# Autodesk Inventor assembly: MechanumChassis
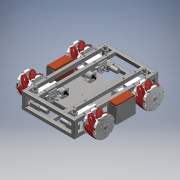
[picture p0: Inventor's stored thumbnail of the model, 180x180]
Saved by Autodesk Inventor 2018 (Build 220112000, 112)
## iProperties
Created: 2017-10-18
Part Number: MechanumChassis
Document SubType Name: Weldment
Designer: Bryce Richards
Mass: 42172.1 g
Surface Area: 44852.8 cm^2
Volume: 5448.29 cm^3
Density: 7.74044 g/cm^3
Weld Material: Steel, Mild, Welded
Author: Bryce Richards
## Documents named in this file (16)
- C:\Users\P136265\Documents\GitHub\mecanum-cad\MechanumChassis.iam
- C:\Users\P136265\Documents\GitHub\mecanum-cad\MecanumFrame2.iam
- C:\Users\P136265\Documents\GitHub\mecanum-cad\WheelShaft.ipt
- C:\Users\P136265\Documents\GitHub\mecanum-cad\Mecanum_Assembly.iam
- C:\Users\P136265\Documents\Inventor\Content Center Files\R2018\en-US\AS 1112 (2)\AS 1112 - M4  Type 5.ipt
- C:\Users\P136265\Documents\GitHub\mecanum-cad\LiftBase.ipt
- C:\Users\P136265\Documents\GitHub\mecanum-cad\BatteryBox_NP1812.ipt
- C:\Users\P136265\Documents\GitHub\mecanum-cad\NP18-12 Battery.ipt
- C:\Users\P136265\Documents\GitHub\mecanum-cad\BearingHousing.iam
- C:\Users\P136265\Documents\Inventor\Content Center Files\R2018\en-US\AS 1110\AS 1110 - M8 x 50.ipt
- C:\Users\P136265\Documents\Inventor\Content Center Files\R2018\en-US\AS 1112 (2)\AS 1112 - M8  Type 5.ipt
- C:\Users\P136265\Documents\GitHub\mecanum-cad\mount.ipt
- C:\Users\P136265\Documents\GitHub\mecanum-cad\Nema 23 Stepper Motor Bipolar L=56mm w Gear Ratio 41 Planetary Gearbox.ipt
- C:\Users\P136265\Documents\GitHub\mecanum-cad\LiftAssembly_Through.iam
- C:\Users\P136265\Documents\Inventor\Content Center Files\R2018\en-US\BS EN 24035\ISO 4035 - M20BS EN.ipt
- C:\Users\P136265\Documents\mecanum-cad\MechanumChassis\AIP\FEA\cayefugld.fres
## Components (78 placed, 14 different names)
1. MecanumFrame2:1 [sub-assembly] — Mate:90, Angle:5, Angle:6, Angle:7, Mate:386, Flush:32, Flush:33, Mate:486, Mate:487, Mate:488, Mate:489, Mate:494, Mate:500, Mate:501, Mate:502, Mate:503, Mate:504, Mate:512, Mate:514, Mate:516, Mate:518, Mate:520, Mate:522, Mate:524, Mate:526, Mate:528, Mate:530, Mate:532, Mate:534, Mate:536, Mate:538, Mate:540, Mate:542, Mate:545, Mate:547, Mate:549, Mate:551, Mate:553, Mate:555, Mate:557, Mate:559, Mate:561, Mate:563, Mate:565, Mate:567, Mate:569, Mate:571, Mate:573, Mate:575, Mate:594, Angle:41, Mate:607, Mate:608, Mate:641, Mate:642, Mate:643, Mate:644, Mate:645, Mate:646, Angle:49, Angle:51
2. Mecanum_Assembly:1 [sub-assembly] — Mate:617, Mate:618, Angle:44, Mate:654
3. Mecanum_Assembly:2 [sub-assembly] — Mate:613, Mate:614, Angle:43, Mate:652
4. Mecanum_Assembly:3 [sub-assembly] — Mate:621, Mate:622, Mate:650
5. Mecanum_Assembly:4 [sub-assembly] — Mate:609, Mate:610, Angle:42, Mate:648
6. LiftBase:1 — Mate:386, Flush:32, Flush:33, Mate:606, Mate:635, Mate:637, Mate:639
7. BatteryBox_NP1812:1 — Mate:459, Mate:461
8. BatteryBox_NP1812:2 — Mate:462, Mate:464
9. NP18-12 Battery:1 — Mate:459, Mate:461, Angle:45, Angle:46
10. NP18-12 Battery:2 — Mate:462, Mate:464, Angle:40, Angle:47
11. AS 1112 (2) - Metric M4  Type 5:17
12. AS 1112 (2) - Metric M4  Type 5:18
13. AS 1112 (2) - Metric M4  Type 5:19
14. AS 1112 (2) - Metric M4  Type 5:20
15. AS 1112 (2) - Metric M4  Type 5:21
16. AS 1112 (2) - Metric M4  Type 5:22
17. AS 1112 (2) - Metric M4  Type 5:23
18. AS 1112 (2) - Metric M4  Type 5:24
19. BearingHousing:1 [sub-assembly] — Mate:486, Mate:487, Mate:488, Mate:489, Mate:493, Mate:521, Mate:523, Mate:525, Mate:527, Mate:611, Mate:612, Mate:660
20. BearingHousing:2 [sub-assembly] — Mate:493, Mate:494, Mate:513, Mate:515, Mate:517, Mate:519, Mate:594, Mate:615, Mate:616, Mate:658
21. BearingHousing:3 [sub-assembly] — Mate:503, Mate:504, Mate:529, Mate:531, Mate:533, Mate:535, Mate:623, Mate:624, Mate:662
22. BearingHousing:4 [sub-assembly] — Mate:500, Mate:501, Mate:502, Mate:537, Mate:539, Mate:541, Mate:543, Mate:619, Mate:620, Mate:656
23. AS 1110 - Metric M8 x 50:3 — Mate:512, Mate:513, Mate:558
24. AS 1110 - Metric M8 x 50:4 — Mate:514, Mate:515, Mate:556
25. AS 1110 - Metric M8 x 50:5 — Mate:516, Mate:517, Mate:552
26. AS 1110 - Metric M8 x 50:6 — Mate:518, Mate:519, Mate:554
27. AS 1110 - Metric M8 x 50:7 — Mate:520, Mate:521, Mate:574
28. AS 1110 - Metric M8 x 50:8 — Mate:522, Mate:523, Mate:572
29. AS 1110 - Metric M8 x 50:9 — Mate:524, Mate:525, Mate:568
30. AS 1110 - Metric M8 x 50:10 — Mate:526, Mate:527, Mate:570
31. AS 1110 - Metric M8 x 50:11 — Mate:528, Mate:529, Mate:566
32. AS 1110 - Metric M8 x 50:12 — Mate:530, Mate:531, Mate:562
33. AS 1110 - Metric M8 x 50:13 — Mate:532, Mate:533, Mate:564
34. AS 1110 - Metric M8 x 50:14 — Mate:534, Mate:535, Mate:560
35. AS 1110 - Metric M8 x 50:15 — Mate:536, Mate:537, Mate:544
36. AS 1110 - Metric M8 x 50:16 — Mate:538, Mate:539, Mate:548
37. AS 1110 - Metric M8 x 50:17 — Mate:540, Mate:541, Mate:546
38. AS 1110 - Metric M8 x 50:18 — Mate:542, Mate:543, Mate:550
39. AS 1112 (2) - Metric M8  Type 5:1 — Mate:544, Mate:545
40. AS 1112 (2) - Metric M8  Type 5:2 — Mate:546, Mate:547
41. AS 1112 (2) - Metric M8  Type 5:3 — Mate:548, Mate:549
42. AS 1112 (2) - Metric M8  Type 5:4 — Mate:550, Mate:551
43. AS 1112 (2) - Metric M8  Type 5:5 — Mate:552, Mate:553
44. AS 1112 (2) - Metric M8  Type 5:6 — Mate:554, Mate:555
45. AS 1112 (2) - Metric M8  Type 5:7 — Mate:556, Mate:557
46. AS 1112 (2) - Metric M8  Type 5:8 — Mate:558, Mate:559
47. AS 1112 (2) - Metric M8  Type 5:9 — Mate:560, Mate:561
48. AS 1112 (2) - Metric M8  Type 5:10 — Mate:562, Mate:563
49. AS 1112 (2) - Metric M8  Type 5:11 — Mate:564, Mate:565
50. AS 1112 (2) - Metric M8  Type 5:12 — Mate:566, Mate:567
51. AS 1112 (2) - Metric M8  Type 5:13 — Mate:568, Mate:569
52. AS 1112 (2) - Metric M8  Type 5:14 — Mate:570, Mate:571
53. AS 1112 (2) - Metric M8  Type 5:15 — Mate:572, Mate:573
54. AS 1112 (2) - Metric M8  Type 5:16 — Mate:574, Mate:575
55. mount:1 — Mate:603, Mate:604, Mate:605, Mate:606
56. Nema 23 Stepper Motor Bipolar L=56mm w Gear Ratio 41 Planetary Gearbox:1 — Mate:603, Mate:604, Mate:605, Angle:40, Angle:41, Flush:34, Mate:625
57. LiftAssembly_Through:1 [sub-assembly] — Mate:607, Mate:608, Angle:48
58. WheelShaft:1 — Mate:621, Mate:622, Mate:623, Mate:624, Flush:37, Mate:640, Mate:649, Mate:661
59. WheelShaft:2 — Mate:617, Mate:618, Mate:619, Mate:620, Angle:44, Flush:36, Mate:638, Mate:653, Mate:655
60. WheelShaft:3 — Mate:613, Mate:614, Mate:615, Mate:616, Angle:43, Flush:35, Mate:636, Mate:651, Mate:657
61. WheelShaft:4 — Mate:609, Mate:610, Angle:42, Mate:611, Mate:612, Flush:34, Mate:625, Mate:647, Mate:659
62. mount:2 — Mate:626, Mate:627, Mate:628, Mate:637
63. mount:3 — Mate:629, Mate:630, Mate:631, Mate:639
64. mount:4 — Mate:632, Mate:633, Mate:634, Mate:635
65. Nema 23 Stepper Motor Bipolar L=56mm w Gear Ratio 41 Planetary Gearbox:2 — Mate:626, Mate:627, Mate:628, Angle:46, Flush:36, Mate:638
66. Nema 23 Stepper Motor Bipolar L=56mm w Gear Ratio 41 Planetary Gearbox:3 — Mate:629, Mate:630, Mate:631, Angle:47, Flush:37, Mate:640
67. Nema 23 Stepper Motor Bipolar L=56mm w Gear Ratio 41 Planetary Gearbox:4 — Mate:632, Mate:633, Mate:634, Angle:45, Flush:35, Mate:636
68. LiftAssembly_Through:2 [sub-assembly] — Mate:641, Mate:642, Angle:50, Angle:51
69. LiftAssembly_Through:3 [sub-assembly] — Mate:643, Mate:644, Angle:50
70. LiftAssembly_Through:4 [sub-assembly] — Mate:645, Mate:646, Angle:48, Angle:49
71. BS EN 24035 - Metric M20:1 — Mate:647, Mate:648
72. BS EN 24035 - Metric M20:2 — Mate:649, Mate:650
73. BS EN 24035 - Metric M20:3 — Mate:651, Mate:652
74. BS EN 24035 - Metric M20:4 — Mate:653, Mate:654
75. BS EN 24035 - Metric M20:5 — Mate:655, Mate:656
76. BS EN 24035 - Metric M20:6 — Mate:657, Mate:658
77. BS EN 24035 - Metric M20:7 — Mate:659, Mate:660
78. BS EN 24035 - Metric M20:8 — Mate:661, Mate:662
## Relationships (163: Mate 142, Angle 15, Flush 6)
- Mate:90: MecanumFrame2:1
- Angle:5 (0 deg): MecanumFrame2:1
- Angle:6 (0 deg): MecanumFrame2:1
- Angle:7 (0 deg): MecanumFrame2:1
- Mate:386: MecanumFrame2:1 ↔ LiftBase:1
- Flush:32 (2.5 mm): MecanumFrame2:1 ↔ LiftBase:1
- Flush:33 (2.5 mm): MecanumFrame2:1 ↔ LiftBase:1
- Mate:459: BatteryBox_NP1812:1 ↔ NP18-12 Battery:1
- Mate:461 (2 mm): BatteryBox_NP1812:1 ↔ NP18-12 Battery:1
- Mate:462: BatteryBox_NP1812:2 ↔ NP18-12 Battery:2
- Mate:464 (2 mm): BatteryBox_NP1812:2 ↔ NP18-12 Battery:2
- Mate:486: MecanumFrame2:1 ↔ BearingHousing:1
- Mate:487: MecanumFrame2:1 ↔ BearingHousing:1
- Mate:488: MecanumFrame2:1 ↔ BearingHousing:1
- Mate:489: MecanumFrame2:1 ↔ BearingHousing:1
- Mate:493: BearingHousing:1 ↔ BearingHousing:2
- Mate:494: MecanumFrame2:1 ↔ BearingHousing:2
- Mate:500: MecanumFrame2:1 ↔ BearingHousing:4
- Mate:501: MecanumFrame2:1 ↔ BearingHousing:4
- Mate:502: MecanumFrame2:1 ↔ BearingHousing:4
- Mate:503: MecanumFrame2:1 ↔ BearingHousing:3
- Mate:504: MecanumFrame2:1 ↔ BearingHousing:3
- Mate:512: MecanumFrame2:1 ↔ AS 1110 - Metric M8 x 50:3
- Mate:513: BearingHousing:2 ↔ AS 1110 - Metric M8 x 50:3
- Mate:514: MecanumFrame2:1 ↔ AS 1110 - Metric M8 x 50:4
- Mate:515: BearingHousing:2 ↔ AS 1110 - Metric M8 x 50:4
- Mate:516: MecanumFrame2:1 ↔ AS 1110 - Metric M8 x 50:5
- Mate:517: BearingHousing:2 ↔ AS 1110 - Metric M8 x 50:5
- Mate:518: MecanumFrame2:1 ↔ AS 1110 - Metric M8 x 50:6
- Mate:519: BearingHousing:2 ↔ AS 1110 - Metric M8 x 50:6
- Mate:520: MecanumFrame2:1 ↔ AS 1110 - Metric M8 x 50:7
- Mate:521: BearingHousing:1 ↔ AS 1110 - Metric M8 x 50:7
- Mate:522: MecanumFrame2:1 ↔ AS 1110 - Metric M8 x 50:8
- Mate:523: BearingHousing:1 ↔ AS 1110 - Metric M8 x 50:8
- Mate:524: MecanumFrame2:1 ↔ AS 1110 - Metric M8 x 50:9
- Mate:525: BearingHousing:1 ↔ AS 1110 - Metric M8 x 50:9
- Mate:526: MecanumFrame2:1 ↔ AS 1110 - Metric M8 x 50:10
- Mate:527: BearingHousing:1 ↔ AS 1110 - Metric M8 x 50:10
- Mate:528: MecanumFrame2:1 ↔ AS 1110 - Metric M8 x 50:11
- Mate:529: BearingHousing:3 ↔ AS 1110 - Metric M8 x 50:11
- Mate:530: MecanumFrame2:1 ↔ AS 1110 - Metric M8 x 50:12
- Mate:531: BearingHousing:3 ↔ AS 1110 - Metric M8 x 50:12
- Mate:532: MecanumFrame2:1 ↔ AS 1110 - Metric M8 x 50:13
- Mate:533: BearingHousing:3 ↔ AS 1110 - Metric M8 x 50:13
- Mate:534: MecanumFrame2:1 ↔ AS 1110 - Metric M8 x 50:14
- Mate:535: BearingHousing:3 ↔ AS 1110 - Metric M8 x 50:14
- Mate:536: MecanumFrame2:1 ↔ AS 1110 - Metric M8 x 50:15
- Mate:537: BearingHousing:4 ↔ AS 1110 - Metric M8 x 50:15
- Mate:538: MecanumFrame2:1 ↔ AS 1110 - Metric M8 x 50:16
- Mate:539: BearingHousing:4 ↔ AS 1110 - Metric M8 x 50:16
- Mate:540: MecanumFrame2:1 ↔ AS 1110 - Metric M8 x 50:17
- Mate:541: BearingHousing:4 ↔ AS 1110 - Metric M8 x 50:17
- Mate:542: MecanumFrame2:1 ↔ AS 1110 - Metric M8 x 50:18
- Mate:543: BearingHousing:4 ↔ AS 1110 - Metric M8 x 50:18
- Mate:544: AS 1110 - Metric M8 x 50:15 ↔ AS 1112 (2) - Metric M8  Type 5:1
- Mate:545: MecanumFrame2:1 ↔ AS 1112 (2) - Metric M8  Type 5:1
- Mate:546: AS 1110 - Metric M8 x 50:17 ↔ AS 1112 (2) - Metric M8  Type 5:2
- Mate:547: MecanumFrame2:1 ↔ AS 1112 (2) - Metric M8  Type 5:2
- Mate:548: AS 1110 - Metric M8 x 50:16 ↔ AS 1112 (2) - Metric M8  Type 5:3
- Mate:549: MecanumFrame2:1 ↔ AS 1112 (2) - Metric M8  Type 5:3
- Mate:550: AS 1110 - Metric M8 x 50:18 ↔ AS 1112 (2) - Metric M8  Type 5:4
- Mate:551: MecanumFrame2:1 ↔ AS 1112 (2) - Metric M8  Type 5:4
- Mate:552: AS 1110 - Metric M8 x 50:5 ↔ AS 1112 (2) - Metric M8  Type 5:5
- Mate:553: MecanumFrame2:1 ↔ AS 1112 (2) - Metric M8  Type 5:5
- Mate:554: AS 1110 - Metric M8 x 50:6 ↔ AS 1112 (2) - Metric M8  Type 5:6
- Mate:555: MecanumFrame2:1 ↔ AS 1112 (2) - Metric M8  Type 5:6
- Mate:556: AS 1110 - Metric M8 x 50:4 ↔ AS 1112 (2) - Metric M8  Type 5:7
- Mate:557: MecanumFrame2:1 ↔ AS 1112 (2) - Metric M8  Type 5:7
- Mate:558: AS 1110 - Metric M8 x 50:3 ↔ AS 1112 (2) - Metric M8  Type 5:8
- Mate:559: MecanumFrame2:1 ↔ AS 1112 (2) - Metric M8  Type 5:8
- Mate:560: AS 1110 - Metric M8 x 50:14 ↔ AS 1112 (2) - Metric M8  Type 5:9
- Mate:561: MecanumFrame2:1 ↔ AS 1112 (2) - Metric M8  Type 5:9
- Mate:562: AS 1110 - Metric M8 x 50:12 ↔ AS 1112 (2) - Metric M8  Type 5:10
- Mate:563: MecanumFrame2:1 ↔ AS 1112 (2) - Metric M8  Type 5:10
- Mate:564: AS 1110 - Metric M8 x 50:13 ↔ AS 1112 (2) - Metric M8  Type 5:11
- Mate:565: MecanumFrame2:1 ↔ AS 1112 (2) - Metric M8  Type 5:11
- Mate:566: AS 1110 - Metric M8 x 50:11 ↔ AS 1112 (2) - Metric M8  Type 5:12
- Mate:567: MecanumFrame2:1 ↔ AS 1112 (2) - Metric M8  Type 5:12
- Mate:568: AS 1110 - Metric M8 x 50:9 ↔ AS 1112 (2) - Metric M8  Type 5:13
- Mate:569: MecanumFrame2:1 ↔ AS 1112 (2) - Metric M8  Type 5:13
- Mate:570: AS 1110 - Metric M8 x 50:10 ↔ AS 1112 (2) - Metric M8  Type 5:14
- Mate:571: MecanumFrame2:1 ↔ AS 1112 (2) - Metric M8  Type 5:14
- Mate:572: AS 1110 - Metric M8 x 50:8 ↔ AS 1112 (2) - Metric M8  Type 5:15
- Mate:573: MecanumFrame2:1 ↔ AS 1112 (2) - Metric M8  Type 5:15
- Mate:574: AS 1110 - Metric M8 x 50:7 ↔ AS 1112 (2) - Metric M8  Type 5:16
- Mate:575: MecanumFrame2:1 ↔ AS 1112 (2) - Metric M8  Type 5:16
- Mate:594: MecanumFrame2:1 ↔ BearingHousing:2
- Mate:603: mount:1 ↔ Nema 23 Stepper Motor Bipolar L=56mm w Gear Ratio 41 Planetary Gearbox:1
- Mate:604: mount:1 ↔ Nema 23 Stepper Motor Bipolar L=56mm w Gear Ratio 41 Planetary Gearbox:1
- Mate:605: mount:1 ↔ Nema 23 Stepper Motor Bipolar L=56mm w Gear Ratio 41 Planetary Gearbox:1
- Mate:606: LiftBase:1 ↔ mount:1
- Angle:40 (180 deg): NP18-12 Battery:2 ↔ Nema 23 Stepper Motor Bipolar L=56mm w Gear Ratio 41 Planetary Gearbox:1
- Angle:41 (0 deg): MecanumFrame2:1 ↔ Nema 23 Stepper Motor Bipolar L=56mm w Gear Ratio 41 Planetary Gearbox:1
- Mate:607: MecanumFrame2:1 ↔ LiftAssembly_Through:1
- Mate:608: MecanumFrame2:1 ↔ LiftAssembly_Through:1
- Mate:609: Mecanum_Assembly:4 ↔ WheelShaft:4
- Mate:610: Mecanum_Assembly:4 ↔ WheelShaft:4
- Angle:42 (0 deg): Mecanum_Assembly:4 ↔ WheelShaft:4
- Mate:611: BearingHousing:1 ↔ WheelShaft:4
- Mate:612: BearingHousing:1 ↔ WheelShaft:4
- Flush:34 (10 mm): Nema 23 Stepper Motor Bipolar L=56mm w Gear Ratio 41 Planetary Gearbox:1 ↔ WheelShaft:4
- Mate:613: Mecanum_Assembly:2 ↔ WheelShaft:3
- Mate:614: Mecanum_Assembly:2 ↔ WheelShaft:3
- Mate:615: BearingHousing:2 ↔ WheelShaft:3
- Mate:616: BearingHousing:2 ↔ WheelShaft:3
- Angle:43 (0 deg): Mecanum_Assembly:2 ↔ WheelShaft:3
- Mate:617: Mecanum_Assembly:1 ↔ WheelShaft:2
- Mate:618: Mecanum_Assembly:1 ↔ WheelShaft:2
- Mate:619: BearingHousing:4 ↔ WheelShaft:2
- Mate:620: BearingHousing:4 ↔ WheelShaft:2
- Angle:44 (0 deg): Mecanum_Assembly:1 ↔ WheelShaft:2
- Mate:621: Mecanum_Assembly:3 ↔ WheelShaft:1
- Mate:622: Mecanum_Assembly:3 ↔ WheelShaft:1
- Mate:623: BearingHousing:3 ↔ WheelShaft:1
- Mate:624: BearingHousing:3 ↔ WheelShaft:1
- Mate:625 (107.5 mm): Nema 23 Stepper Motor Bipolar L=56mm w Gear Ratio 41 Planetary Gearbox:1 ↔ WheelShaft:4
- Mate:626: mount:2 ↔ Nema 23 Stepper Motor Bipolar L=56mm w Gear Ratio 41 Planetary Gearbox:2
- Mate:627: mount:2 ↔ Nema 23 Stepper Motor Bipolar L=56mm w Gear Ratio 41 Planetary Gearbox:2
- Mate:628: mount:2 ↔ Nema 23 Stepper Motor Bipolar L=56mm w Gear Ratio 41 Planetary Gearbox:2
- Mate:629: mount:3 ↔ Nema 23 Stepper Motor Bipolar L=56mm w Gear Ratio 41 Planetary Gearbox:3
- Mate:630: mount:3 ↔ Nema 23 Stepper Motor Bipolar L=56mm w Gear Ratio 41 Planetary Gearbox:3
- Mate:631: mount:3 ↔ Nema 23 Stepper Motor Bipolar L=56mm w Gear Ratio 41 Planetary Gearbox:3
- Mate:632: mount:4 ↔ Nema 23 Stepper Motor Bipolar L=56mm w Gear Ratio 41 Planetary Gearbox:4
- Mate:633: mount:4 ↔ Nema 23 Stepper Motor Bipolar L=56mm w Gear Ratio 41 Planetary Gearbox:4
- Mate:634: mount:4 ↔ Nema 23 Stepper Motor Bipolar L=56mm w Gear Ratio 41 Planetary Gearbox:4
- Mate:635: LiftBase:1 ↔ mount:4
- Angle:45 (0 deg): NP18-12 Battery:1 ↔ Nema 23 Stepper Motor Bipolar L=56mm w Gear Ratio 41 Planetary Gearbox:4
- Flush:35 (10 mm): WheelShaft:3 ↔ Nema 23 Stepper Motor Bipolar L=56mm w Gear Ratio 41 Planetary Gearbox:4
- Mate:636 (107.5 mm): WheelShaft:3 ↔ Nema 23 Stepper Motor Bipolar L=56mm w Gear Ratio 41 Planetary Gearbox:4
- Mate:637: LiftBase:1 ↔ mount:2
- Angle:46 (0 deg): NP18-12 Battery:1 ↔ Nema 23 Stepper Motor Bipolar L=56mm w Gear Ratio 41 Planetary Gearbox:2
- Flush:36 (10 mm): WheelShaft:2 ↔ Nema 23 Stepper Motor Bipolar L=56mm w Gear Ratio 41 Planetary Gearbox:2
- Mate:638 (107.5 mm): WheelShaft:2 ↔ Nema 23 Stepper Motor Bipolar L=56mm w Gear Ratio 41 Planetary Gearbox:2
- Angle:47 (0 deg): NP18-12 Battery:2 ↔ Nema 23 Stepper Motor Bipolar L=56mm w Gear Ratio 41 Planetary Gearbox:3
- Mate:639: LiftBase:1 ↔ mount:3
- Flush:37 (10 mm): WheelShaft:1 ↔ Nema 23 Stepper Motor Bipolar L=56mm w Gear Ratio 41 Planetary Gearbox:3
- Mate:640 (107.5 mm): WheelShaft:1 ↔ Nema 23 Stepper Motor Bipolar L=56mm w Gear Ratio 41 Planetary Gearbox:3
- Mate:641: MecanumFrame2:1 ↔ LiftAssembly_Through:2
- Mate:642: MecanumFrame2:1 ↔ LiftAssembly_Through:2
- Mate:643: MecanumFrame2:1 ↔ LiftAssembly_Through:3
- Mate:644: MecanumFrame2:1 ↔ LiftAssembly_Through:3
- Mate:645: MecanumFrame2:1 ↔ LiftAssembly_Through:4
- Mate:646: MecanumFrame2:1 ↔ LiftAssembly_Through:4
- Angle:48 (0 deg): LiftAssembly_Through:1 ↔ LiftAssembly_Through:4
- Angle:49 (0 deg): MecanumFrame2:1 ↔ LiftAssembly_Through:4
- Angle:50 (0 deg): LiftAssembly_Through:2 ↔ LiftAssembly_Through:3
- Angle:51 (0 deg): MecanumFrame2:1 ↔ LiftAssembly_Through:2
- Mate:647: WheelShaft:4 ↔ BS EN 24035 - Metric M20:1
- Mate:648: Mecanum_Assembly:4 ↔ BS EN 24035 - Metric M20:1
- Mate:649: WheelShaft:1 ↔ BS EN 24035 - Metric M20:2
- Mate:650: Mecanum_Assembly:3 ↔ BS EN 24035 - Metric M20:2
- Mate:651: WheelShaft:3 ↔ BS EN 24035 - Metric M20:3
- Mate:652: Mecanum_Assembly:2 ↔ BS EN 24035 - Metric M20:3
- Mate:653: WheelShaft:2 ↔ BS EN 24035 - Metric M20:4
- Mate:654: Mecanum_Assembly:1 ↔ BS EN 24035 - Metric M20:4
- Mate:655: WheelShaft:2 ↔ BS EN 24035 - Metric M20:5
- Mate:656: BearingHousing:4 ↔ BS EN 24035 - Metric M20:5
- Mate:657: WheelShaft:3 ↔ BS EN 24035 - Metric M20:6
- Mate:658: BearingHousing:2 ↔ BS EN 24035 - Metric M20:6
- Mate:659: WheelShaft:4 ↔ BS EN 24035 - Metric M20:7
- Mate:660: BearingHousing:1 ↔ BS EN 24035 - Metric M20:7
- Mate:661: WheelShaft:1 ↔ BS EN 24035 - Metric M20:8
- Mate:662: BearingHousing:3 ↔ BS EN 24035 - Metric M20:8
## Named parameters: sa_0 = 0, sa_1 = -3.88819e-08, sa_2 = 1e+06
note: some values were not read from the file. Shown as the stored number, unit unknown: "sa_0", "sa_1", "sa_2".
